# Autodesk Inventor assembly: MX-28
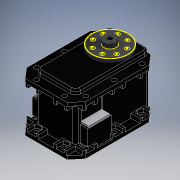
[picture p0: Inventor's stored thumbnail of the model, 180x180]
Saved by Autodesk Inventor 2022 (Build 260153000, 153)
## iProperties
Created: 2020-07-09
Part Number: MX-28
Material: Типовые
Document SubType Name: Assembly
Designer: Петров Иван
Author: Петров Иван
## Documents named in this file (3)
- C:\Users\Ivan Petrov\Documents\GitHub\OmniBot\design\standart_components\dynamixels\mx-28\MX-28.iam
- C:\Users\Ivan Petrov\Documents\GitHub\OmniBot\design\standart_components\dynamixels\mx-28\MX-28T_R.ipt
- C:\Users\Ivan Petrov\Documents\GitHub\OmniBot\design\standart_components\dynamixels\mx-28\Disk_driver_MX28.ipt
## Components (2 placed, 2 different names)
1. MX-28T_R:1 — Mate:1, Mate:2
2. Disk_driver_MX28:1 — Mate:1, Mate:2
## Relationships (2: Mate 2)
- Mate:1: MX-28T_R:1 ↔ Disk_driver_MX28:1
- Mate:2: MX-28T_R:1 ↔ Disk_driver_MX28:1
